# Autodesk Inventor assembly: lightweight carrige v2
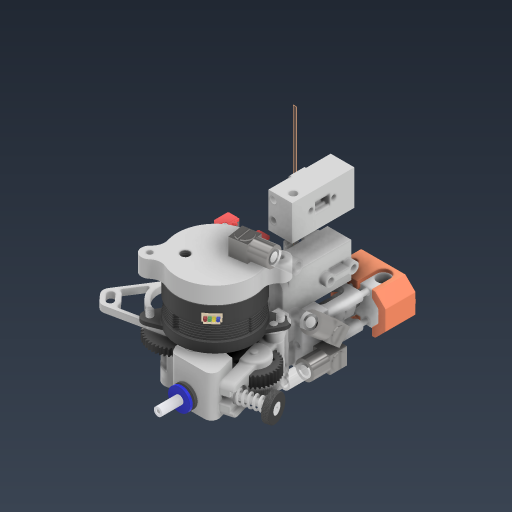
[picture p0: Inventor's stored thumbnail of the model, 512x512]
Saved by Autodesk Inventor 2024.3 (Build 283343000, 343)
## iProperties
Created: 2024-09-28
Part Number: lightweight carrige v2
Document SubType Name: Assembly
Designer: MFil
Author: MFil
## Documents named in this file (30)
- C:\ROBOTYKA\myVORON tridex\Hotend carriges\thin carrige\lightweight carrige v2.iam
- C:\ROBOTYKA\myVORON tridex\Hotend carriges\thin carrige\radiator CNC rev2.ipt
- C:\ROBOTYKA\myVORON tridex\Hotend carriges\thin carrige\MGN9H Block.ipt
- C:\ROBOTYKA\myVORON tridex\Hotend carriges\thin carrige\Idler_arm_MIR.ipt
- C:\ROBOTYKA\myVORON tridex\Hotend carriges\thin carrige\LDO-36STH20-1004AHG.ipt
- C:\ROBOTYKA\myVORON tridex\Hotend carriges\thin carrige\LGX 17T-44T Gear.ipt
- C:\ROBOTYKA\myVORON tridex\Hotend carriges\thin carrige\LGX Hobbed Gear (R).iam
- C:\ROBOTYKA\myVORON tridex\Hotend carriges\thin carrige\MR63ZZ (B).ipt
- C:\ROBOTYKA\myVORON tridex\Hotend carriges\thin carrige\Rocker shaft.ipt
- C:\ROBOTYKA\myVORON tridex\Hotend carriges\thin carrige\Screw M3x8.ipt
- C:\ROBOTYKA\myVORON tridex\Hotend carriges\thin carrige\Rocker screw BASE.iam
- C:\ROBOTYKA\myVORON tridex\Parts\tridex belt a_CPY 4.ipt
- C:\ROBOTYKA\myVORON tridex\Hotend carriges\parts\filament piece.ipt
- C:\ROBOTYKA\myVORON tridex\Parts\IR-endstop-0.4.1.ipt
- C:\ROBOTYKA\myVORON tridex\Hotend carriges\thin carrige\Screw M3x25.ipt
- C:\ROBOTYKA\myVORON tridex\Hotend carriges\thin carrige\block standoffs.ipt
- C:\ROBOTYKA\myVORON tridex\Hotend carriges\thin carrige\block.ipt
- C:\ROBOTYKA\myVORON tridex\Hotend carriges\thin carrige\heatbreak ender 3s1.ipt
- C:\ROBOTYKA\myVORON tridex\Hotend carriges\thin carrige\melt zone extender.ipt
- C:\ROBOTYKA\myVORON tridex\Hotend carriges\thin carrige\V6 Nozzle.ipt
- C:\ROBOTYKA\myVORON tridex\Hotend carriges\parts\6mm hose fitting.ipt
- C:\ROBOTYKA\myVORON tridex\Hotend carriges\parts\ptfe filament guide.ipt
- C:\ROBOTYKA\myVORON tridex\Hotend carriges\parts\colle ptfe guide.ipt
- C:\ROBOTYKA\myVORON tridex\Hotend carriges\parts\mounting plate.ipt
- C:\ROBOTYKA\myVORON tridex\Hotend carriges\parts\belt clip 1.ipt
- C:\ROBOTYKA\myVORON tridex\Hotend carriges\parts\belt clip 1_MIR1.ipt
- C:\ROBOTYKA\myVORON tridex\Hotend carriges\parts\belt clip 2.ipt
- C:\ROBOTYKA\myVORON tridex\Hotend carriges\parts\extruder backplate.ipt
- C:\ROBOTYKA\myVORON tridex\Hotend carriges\parts\extruder front.ipt
- C:\ROBOTYKA\myVORON tridex\Hotend carriges\parts\extruder waterblock.ipt
## Components (36 placed, 29 different names)
1. radiator CNC rev2:1 — Mate:27, Flush:12, Mate:28, Flush:14, Flush:16, Mate:31, Flush:17, Flush:18, Mate:32, Mate:33, Mate:34, Tangent:5, Flush:20, Flush:21, Flush:22, Flush:23, Mate:35, Mate:37, Mate:38, Mate:39, Flush:29, Mate:56, Mate:57, Mate:64
2. MGN9H Block:1 — Flush:14, Flush:23, Mate:35, Mate:36, Tangent:9, Tangent:11, Flush:28, Flush:30, Mate:54, Mate:55
3. Idler_arm_MIR:1 — Tangent:6
4. LGX Hobbed Gear (R):1 [sub-assembly] — Tangent:3, Flush:18, Tangent:5, Mate:42, Flush:26, Tangent:12
5. Rocker shaft:1
6. LGX Hobbed Gear (R):2 [sub-assembly] — Tangent:2, Tangent:4
7. Rocker screw BASE:1 [sub-assembly]
8. tridex belt a_CPY 4:1
9. tridex belt a_CPY 4:2 — Flush:16, Mate:36, Flush:30
10. block standoffs:1 — Mate:28, Mate:37, Mate:38, Mate:39
11. block:1 — Flush:12
12. heatbreak ender 3s1:1 — Mate:27
13. melt zone extender:1
14. V6 Nozzle:1
15. IR-endstop-0.4.1:1 — Tangent:7, Tangent:8, Flush:22, Tangent:10, Mate:47, Tangent:12
16. filament piece:1 — Mate:31, Flush:17, Tangent:2, Tangent:3, Tangent:4, Tangent:7, Tangent:8, Mate:46
17. Screw M3x25:2 — Mate:48, Flush:29
18. LDO-36STH20-1004AHG:1 — Mate:43, Mate:44, Tangent:9, Tangent:11, Mate:48, Mate:49, Mate:50, Flush:35, Mate:68, Mate:69
19. Screw M3x8:1 — Mate:49, Mate:50
20. MR63ZZ (B):1 — Mate:40, Flush:25, Tangent:10
21. LGX 17T-44T Gear:1 — Mate:41, Flush:24, Flush:25, Mate:42, Mate:43, Flush:26
22. MR63ZZ (B):2 — Mate:40, Mate:41, Flush:24, Mate:44
23. 6mm hose fitting:1 — Mate:32, Flush:19, Mate:34, Flush:21
24. 6mm hose fitting:2 — Mate:33, Flush:19
25. ptfe filament guide:1 — Flush:20, Tangent:6
26. colle ptfe guide:1 — Mate:46, Mate:47
27. mounting plate:1 — Flush:28, Mate:51, Mate:54, Mate:55, Mate:56, Mate:57, Mate:60, Mate:61, Mate:62, Mate:63, Flush:33, Flush:34
28. belt clip 1:1 — Mate:51, Mate:63, Mate:64, Flush:32, Mate:65
29. Screw M3x25:4 — Mate:60, Flush:31
30. Screw M3x25:5 — Mate:61, Flush:31, Mate:62
31. belt clip 1_MIR1:1
32. belt clip 2:1 — Flush:32, Mate:65
33. extruder backplate:1 — Flush:33
34. extruder front:1 — Flush:34
35. extruder waterblock:1 — Flush:35, Mate:66, Mate:67, Mate:68, Mate:69
36. 6mm hose fitting:3 — Mate:66, Mate:67
## Relationships (87: Mate 50, Flush 25, Tangent 12)
- [Mate]: Idler_arm_MIR:1 ↔ Rocker screw BASE:1
- [Mate]: Idler_arm_MIR:1 ↔ Rocker screw BASE:1
- [Flush]: tridex belt a_CPY 4:1 ↔ tridex belt a_CPY 4:2
- [Mate] (2.5 mm): tridex belt a_CPY 4:1 ↔ tridex belt a_CPY 4:2
- [Flush]: tridex belt a_CPY 4:1 ↔ tridex belt a_CPY 4:2
- [Mate] (18.5 mm): LGX Hobbed Gear (R):1 ↔ LGX Hobbed Gear (R):2
- [Mate] (0.4 mm): Idler_arm_MIR:1 ↔ LGX Hobbed Gear (R):2
- [Mate]: Idler_arm_MIR:1 ↔ LGX Hobbed Gear (R):2
- [Flush]: LGX Hobbed Gear (R):1 ↔ LGX Hobbed Gear (R):2
- [Tangent]: LGX Hobbed Gear (R):1 ↔ LGX Hobbed Gear (R):2
- [Mate]: Idler_arm_MIR:1 ↔ Rocker shaft:1
- [Flush] (-4.1 mm): Idler_arm_MIR:1 ↔ Rocker shaft:1
- [Mate]: heatbreak ender 3s1:1 ↔ melt zone extender:1
- [Mate]: heatbreak ender 3s1:1 ↔ melt zone extender:1
- [Mate] (3 mm): block:1 ↔ melt zone extender:1
- [Mate]: melt zone extender:1 ↔ V6 Nozzle:1
- [Mate]: block:1 ↔ melt zone extender:1
- [Mate]: melt zone extender:1 ↔ V6 Nozzle:1
- [Mate]: block standoffs:1 ↔ block:1
- Mate:27: radiator CNC rev2:1 ↔ heatbreak ender 3s1:1
- Flush:12: radiator CNC rev2:1 ↔ block:1
- Mate:28: radiator CNC rev2:1 ↔ block standoffs:1
- Flush:14: radiator CNC rev2:1 ↔ MGN9H Block:1
- Flush:16 (5 mm): radiator CNC rev2:1 ↔ tridex belt a_CPY 4:2
- Mate:31: radiator CNC rev2:1 ↔ filament piece:1
- Flush:17 (60 mm): radiator CNC rev2:1 ↔ filament piece:1
- Tangent:2 (-0.625 mm): LGX Hobbed Gear (R):2 ↔ filament piece:1
- Tangent:3 (-0.625 mm): LGX Hobbed Gear (R):1 ↔ filament piece:1
- Tangent:4 (-8.375 mm): LGX Hobbed Gear (R):2 ↔ filament piece:1
- Flush:18 (-20 mm): radiator CNC rev2:1 ↔ LGX Hobbed Gear (R):1
- Mate:32: radiator CNC rev2:1 ↔ 6mm hose fitting:1
- Mate:33: radiator CNC rev2:1 ↔ 6mm hose fitting:2
- Flush:19: 6mm hose fitting:1 ↔ 6mm hose fitting:2
- Mate:34 (0.5 mm): radiator CNC rev2:1 ↔ 6mm hose fitting:1
- Tangent:5 (15 mm): radiator CNC rev2:1 ↔ LGX Hobbed Gear (R):1
- Flush:20: radiator CNC rev2:1 ↔ ptfe filament guide:1
- Tangent:6 (1 mm): Idler_arm_MIR:1 ↔ ptfe filament guide:1
- Flush:21: radiator CNC rev2:1 ↔ 6mm hose fitting:1
- Tangent:7 (0.525 mm): IR-endstop-0.4.1:1 ↔ filament piece:1
- Tangent:8 (0.075 mm): IR-endstop-0.4.1:1 ↔ filament piece:1
- Flush:22: radiator CNC rev2:1 ↔ IR-endstop-0.4.1:1
- Flush:23: radiator CNC rev2:1 ↔ MGN9H Block:1
- Mate:35 (6 mm): radiator CNC rev2:1 ↔ MGN9H Block:1
- Mate:36 (3.3 mm): MGN9H Block:1 ↔ tridex belt a_CPY 4:2
- Mate:37: radiator CNC rev2:1 ↔ block standoffs:1
- Mate:38: radiator CNC rev2:1 ↔ block standoffs:1
- Mate:39: radiator CNC rev2:1 ↔ block standoffs:1
- Mate:40: MR63ZZ (B):1 ↔ MR63ZZ (B):2
- Mate:41: LGX 17T-44T Gear:1 ↔ MR63ZZ (B):2
- Flush:24: LGX 17T-44T Gear:1 ↔ MR63ZZ (B):2
- Flush:25: MR63ZZ (B):1 ↔ LGX 17T-44T Gear:1
- Mate:42 (13.5 mm): LGX Hobbed Gear (R):1 ↔ LGX 17T-44T Gear:1
- Mate:43 (13.5 mm): LDO-36STH20-1004AHG:1 ↔ LGX 17T-44T Gear:1
- Flush:26: LGX Hobbed Gear (R):1 ↔ LGX 17T-44T Gear:1
- Mate:44 (0.1 mm): LDO-36STH20-1004AHG:1 ↔ MR63ZZ (B):2
- Tangent:9 (6 mm): MGN9H Block:1 ↔ LDO-36STH20-1004AHG:1
- Tangent:10 (2 mm): IR-endstop-0.4.1:1 ↔ MR63ZZ (B):1
- Tangent:11 (6 mm): MGN9H Block:1 ↔ LDO-36STH20-1004AHG:1
- Mate:46: filament piece:1 ↔ colle ptfe guide:1
- Mate:47 (1 mm): IR-endstop-0.4.1:1 ↔ colle ptfe guide:1
- Tangent:12 (10 mm): LGX Hobbed Gear (R):1 ↔ IR-endstop-0.4.1:1
- Flush:28: MGN9H Block:1 ↔ mounting plate:1
- Mate:48: Screw M3x25:2 ↔ LDO-36STH20-1004AHG:1
- Flush:29: radiator CNC rev2:1 ↔ Screw M3x25:2
- Mate:49: LDO-36STH20-1004AHG:1 ↔ Screw M3x8:1
- Mate:50 (3 mm): LDO-36STH20-1004AHG:1 ↔ Screw M3x8:1
- Flush:30 (10.831 mm): MGN9H Block:1 ↔ tridex belt a_CPY 4:2
- Mate:51: mounting plate:1 ↔ belt clip 1:1
- Mate:54: MGN9H Block:1 ↔ mounting plate:1
- Mate:55: MGN9H Block:1 ↔ mounting plate:1
- Mate:56: radiator CNC rev2:1 ↔ mounting plate:1
- Mate:57: radiator CNC rev2:1 ↔ mounting plate:1
- Mate:60: mounting plate:1 ↔ Screw M3x25:4
- Mate:61: mounting plate:1 ↔ Screw M3x25:5
- Flush:31: Screw M3x25:4 ↔ Screw M3x25:5
- Mate:62: mounting plate:1 ↔ Screw M3x25:5
- Mate:63: mounting plate:1 ↔ belt clip 1:1
- Mate:64 (0.5 mm): radiator CNC rev2:1 ↔ belt clip 1:1
- Flush:32: belt clip 1:1 ↔ belt clip 2:1
- Mate:65 (0.2 mm): belt clip 1:1 ↔ belt clip 2:1
- Flush:33: mounting plate:1 ↔ extruder backplate:1
- Flush:34: mounting plate:1 ↔ extruder front:1
- Flush:35: LDO-36STH20-1004AHG:1 ↔ extruder waterblock:1
- Mate:66: extruder waterblock:1 ↔ 6mm hose fitting:3
- Mate:67 (0.5 mm): extruder waterblock:1 ↔ 6mm hose fitting:3
- Mate:68: LDO-36STH20-1004AHG:1 ↔ extruder waterblock:1
- Mate:69: LDO-36STH20-1004AHG:1 ↔ extruder waterblock:1
